# Autodesk Inventor assembly: Intake motor on xrail left
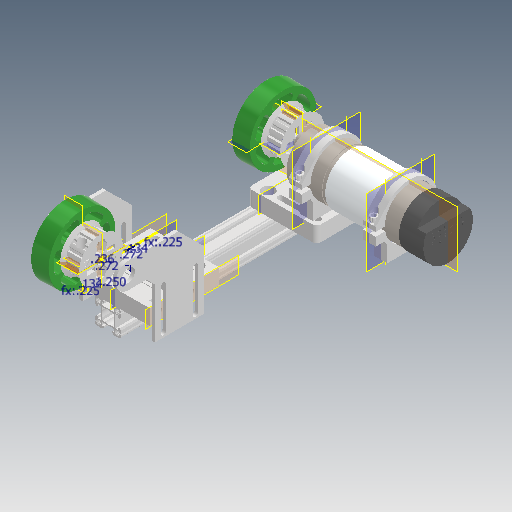
[picture p0: Inventor's stored thumbnail of the model, 512x512]
Saved by Autodesk Inventor 2020 (Build 240168000, 168)
## iProperties
Created: 2020-01-13
Part Number: Intake motor on xrail left
Document SubType Name: Assembly
Designer: ball
Author: ball
## Documents named in this file (6)
- C:\FTC\FTC8863CAD\2019 Robot\Collection\Intake motor on xrail left.iam
- C:\FTC\FTC8863CAD\2019 Robot\Collection\neverest 40 + mounts.iam
- C:\FTC\FTC8863CAD\2019 Robot\Collection\intake motor mount to xrail.ipt
- C:\FTC\FTC8863CAD\Actobotics\565 parts\565030.ipt
- C:\FTC\FTC8863CAD\2019 Robot\general robot componets\pulley .25 in + wheel.2.iam
- C:\FTC\FTC8863CAD\2019 Robot\Collection\Intake\driven wheel assembly.iam
## Components (5 placed, 5 different names)
1. neverest 40 + mounts:1 [sub-assembly] — Flush:3, Flush:5, Mate:5, Mate:6
2. 565030:1 — Flush:6, Mate:7, Flush:7
3. intake motor mount to xrail:1 — Flush:3, Flush:5, Flush:6
4. pulley .25 in + wheel.2:1 [sub-assembly] — Mate:5, Mate:6, Mate:8
5. driven wheel assembly:1 [sub-assembly] — Mate:7, Mate:8, Flush:7
## Relationships (11: Mate 6, Flush 5)
- [Mate]: 565030:1 ↔ intake motor mount to xrail:1
- [Flush]: 565030:1 ↔ intake motor mount to xrail:1
- [Mate]: neverest 40 + mounts:1 ↔ intake motor mount to xrail:1
- Flush:3 (5.08 mm): neverest 40 + mounts:1 ↔ intake motor mount to xrail:1
- Flush:5 (2.3114 mm): neverest 40 + mounts:1 ↔ intake motor mount to xrail:1
- Flush:6: 565030:1 ↔ intake motor mount to xrail:1
- Mate:5: neverest 40 + mounts:1 ↔ pulley .25 in + wheel.2:1
- Mate:6: neverest 40 + mounts:1 ↔ pulley .25 in + wheel.2:1
- Mate:7: 565030:1 ↔ driven wheel assembly:1
- Mate:8: pulley .25 in + wheel.2:1 ↔ driven wheel assembly:1
- Flush:7: 565030:1 ↔ driven wheel assembly:1
